# Autodesk Inventor assembly: ASY TZS 0940 FDS Top elbow
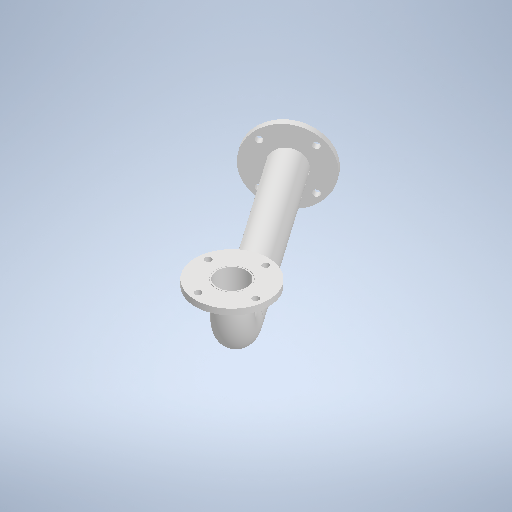
[picture p0: Inventor's stored thumbnail of the model, 512x512]
Saved by Autodesk Inventor 2025 (Build 290162010, 162A)
## iProperties
Created: 2025-07-10
Part Number: ASY TZS 0940 FDS Top elbow
Document SubType Name: Assembly
Designer: user
Author: user
## Documents named in this file (5)
- C:\Users\pokla\Documents\Inventor\TZS-Tazovskiy\Фильтр D940\ASY TZS 0940 FDS Top elbow.iam
- C:\Users\pokla\Documents\Inventor\TZS-Tazovskiy\Фильтр D940\TZS 0942 FDS  tube 1.ipt
- C:\Users\pokla\Documents\Inventor\TZS-Tazovskiy\Фильтр D940\TZS 0941 FDS tube 1.ipt
- C:\Users\pokla\Documents\Inventor\Content Center Files\R2025\en-US\JIS B 2220 SOP - 10K(2)\JIS B 2220 Slip-On Welding Thin Plate Type Flange SOP - 10K 65.ipt
- C:\Users\pokla\Documents\Inventor\Content Center Files\R2025\en-US\JIS B 2312 90 (2)\JIS B 2312 90 Deg Long Elbow Steel 65A x Sch 40.ipt
## Components (5 placed, 4 different names)
1. DIN 2576 Slip-On Flange for Welding Series 1 (ISO) - PN 10 80 x 88.9.ipt:1 — Rigid:7
2. TZS 0941 FDS tube 1.ipt:1 — Rigid:7
3. JIS B 2312 90 Deg Long Elbow Steel 80A x Sch 40.ipt:1
4. TZS 0942 FDS  tube 1.ipt:1 — Rigid:8
5. DIN 2576 Slip-On Flange for Welding Series 1 (ISO) - PN 10 80 x 88.9.ipt:2 — Rigid:8
## Relationships (4: WeldJoint 4)
- [WeldJoint]: TZS 0941 FDS tube 1.ipt:1 ↔ JIS B 2312 90 Deg Long Elbow Steel 80A x Sch 40.ipt:1
- [WeldJoint]: JIS B 2312 90 Deg Long Elbow Steel 80A x Sch 40.ipt:1 ↔ TZS 0942 FDS  tube 1.ipt:1
- Rigid:7 [WeldJoint]: DIN 2576 Slip-On Flange for Welding Series 1 (ISO) - PN 10 80 x 88.9.ipt:1 ↔ TZS 0941 FDS tube 1.ipt:1
- Rigid:8 [WeldJoint]: TZS 0942 FDS  tube 1.ipt:1 ↔ DIN 2576 Slip-On Flange for Welding Series 1 (ISO) - PN 10 80 x 88.9.ipt:2
